# Autodesk Inventor assembly: Bed stand
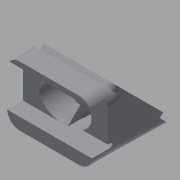
[picture p0: Inventor's stored thumbnail of the model, 180x180]
Saved by Autodesk Inventor 2018 (Build 220112000, 112)
## iProperties
Created: 2020-03-23
Part Number: Bed stand
Document SubType Name: Assembly
Designer: user
Author: user
## Documents named in this file (4)
- D:\Documents\Github\Arduino-MiLightHub_switch\3D\Bed stand.iam
- D:\Documents\Github\Arduino-MiLightHub_switch\3D\V4.ipt
- D:\Documents\Github\Arduino-MiLightHub_switch\3D\V4 In wall.ipt
- D:\Documents\Github\Arduino-MiLightHub_switch\3D\BedStand.ipt
## Components (3 placed, 3 different names)
1. V4:1 — Mate:2, Angle:1
2. V4 In wall:1 — Mate:3, Angle:2
3. BedStand:1 — Mate:2, Angle:1, Mate:3, Angle:2
## Relationships (4: Mate 2, Angle 2)
- Mate:2: V4:1 ↔ BedStand:1
- Angle:1 (0 deg): V4:1 ↔ BedStand:1
- Mate:3: V4 In wall:1 ↔ BedStand:1
- Angle:2 (0 deg): V4 In wall:1 ↔ BedStand:1
